# Autodesk Inventor assembly: base mg996r 3mm with top
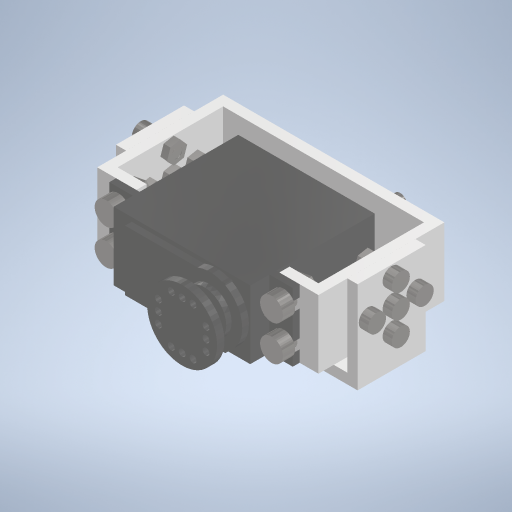
[picture p0: Inventor's stored thumbnail of the model, 512x512]
Saved by Autodesk Inventor 2023 (Build 270158000, 158)
## iProperties
Created: 2022-06-29
Part Number: base mg996r 3mm with top
Document SubType Name: Assembly
Designer: isamu
Author: isamu
## iProperties of the stored document servo frame part 004.ipt
Created: 2022-06-29
Part Number: servo frame part 004
Material: Generic
Document SubType Name: Modeling
Designer: isamu
Density: 1 g/cm^3
Appearance: Default
Author: isamu
## iProperties of the stored document servo frame part 3.iam
Created: 2022-06-29
Part Number: servo frame part 3
Description: FreeCAD Model
Document SubType Name: Assembly
Designer: isamu
Authority: Unknown
Sending System: FreeCAD
Preprocessor: Open CASCADE STEP processor 7.5
Title: Open CASCADE Shape Model
Author: Author
## Documents named in this file (8)
- D:\personal_projects\robot\inventor\base mg996r 3mm with bottom.iam
- **D:\personal_projects\robot\inventor\base mg996r 3mm with bottom.iam*LocalDocs*xAaaaqqaaAaaaaaaaAaaaqcqkKd*servo frame part 3.iam
- D:\personal_projects\robot\inventor\base mg996r 3mm frame.iam
- D:\personal_projects\robot\exports\frames\m3x8.ipt
- D:\personal_projects\robot\exports\frames\m3 nuts.ipt
- **D:\personal_projects\robot\inventor\base mg996r 3mm with top.iam*LocalDocs*xAaaaa3caAaaaaaaaAaaaqro0He*servo frame part 004.ipt
- **D:\personal_projects\robot\inventor\base mg996r 3mm with top.iam*LocalDocs*xAaaaqqaaAaaaaaaaAaaaqcqkKd*servo frame part 3.iam
- D:\personal_projects\robot\exports\frames\servo frame part 3.step
## Components (22 placed, 4 different names)
1. servo frame part 3:1 [sub-assembly] — Mate:2, Insert:1, Insert:3, Insert:4, Insert:5, Insert:11, Insert:12, Insert:13, Insert:14, Insert:15, Mate:3, Mate:4, Insert:21
2. base mg996r 3mm frame:1 [sub-assembly] — Mate:2, Insert:6, Insert:7, Insert:8, Insert:9, Insert:10, Insert:16, Insert:17, Insert:18, Insert:19, Insert:20, Mate:3, Mate:4
3. m3x8:2 — Insert:1
4. m3x8:3 — Insert:5
5. m3x8:4 — Insert:4
6. m3x8:5 — Insert:3
7. m3x8:6 — Insert:11
8. m3x8:7 — Insert:12
9. m3x8:8 — Insert:13
10. m3x8:9 — Insert:14
11. m3x8:10 — Insert:15
12. m3 nuts:1 — Insert:16
13. m3 nuts:2 — Insert:6
14. m3 nuts:3 — Insert:7
15. m3 nuts:4 — Insert:9
16. m3 nuts:5 — Insert:10
17. m3 nuts:6 — Insert:8
18. m3 nuts:7 — Insert:20
19. m3 nuts:8 — Insert:19
20. m3 nuts:9 — Insert:18
21. m3 nuts:10 — Insert:17
22. m3x8:11 — Insert:21
## Relationships (23: Insert 20, Mate 3)
- Mate:2: servo frame part 3:1 ↔ base mg996r 3mm frame:1
- Insert:1: servo frame part 3:1 ↔ m3x8:2
- Insert:3: servo frame part 3:1 ↔ m3x8:5
- Insert:4: servo frame part 3:1 ↔ m3x8:4
- Insert:5: servo frame part 3:1 ↔ m3x8:3
- Insert:6: base mg996r 3mm frame:1 ↔ m3 nuts:2
- Insert:7: base mg996r 3mm frame:1 ↔ m3 nuts:3
- Insert:8: base mg996r 3mm frame:1 ↔ m3 nuts:6
- Insert:9: base mg996r 3mm frame:1 ↔ m3 nuts:4
- Insert:10: base mg996r 3mm frame:1 ↔ m3 nuts:5
- Insert:11: servo frame part 3:1 ↔ m3x8:6
- Insert:12: servo frame part 3:1 ↔ m3x8:7
- Insert:13: servo frame part 3:1 ↔ m3x8:8
- Insert:14: servo frame part 3:1 ↔ m3x8:9
- Insert:15: servo frame part 3:1 ↔ m3x8:10
- Insert:16: base mg996r 3mm frame:1 ↔ m3 nuts:1
- Insert:17: base mg996r 3mm frame:1 ↔ m3 nuts:10
- Insert:18: base mg996r 3mm frame:1 ↔ m3 nuts:9
- Insert:19: base mg996r 3mm frame:1 ↔ m3 nuts:8
- Insert:20: base mg996r 3mm frame:1 ↔ m3 nuts:7
- Mate:3: servo frame part 3:1 ↔ base mg996r 3mm frame:1
- Mate:4: servo frame part 3:1 ↔ base mg996r 3mm frame:1
- Insert:21: servo frame part 3:1 ↔ m3x8:11
